# Autodesk Inventor assembly: 1050.000(1)
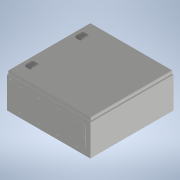
[picture p0: Inventor's stored thumbnail of the model, 180x180]
Saved by Autodesk Inventor 2021 (Build 250183000, 183)
## iProperties
Category: PARTsolutions
Company: RITTAL
Created: 2025-07-29
Part Number: 1050.000(1)
Catalog Web Link: www.cadenas.de
Description: AX Compact enclosure-sheet steel
Vendor: RITTAL
Document SubType Name: Assembly
Designer: psAdmin
Manufacturer: RITTAL
Mass: 2069.6 g
Surface Area: 25440.2 cm^2
Volume: 2069.6 cm^3
Density: 1 g/cm^3
Title: 1050.000(1)
Author: Cadenas PARTsolutions
Comments: sheet steel
PSOL_IDENT_0: {$CADENAS_DATA/23d-libs/rittal/schaltschranksys/kompakt_schaltschr/ae_2_0_asmtab.prj},203 {VTYP=3D},
PSOL_IDENT_1: {STYP=ASSTAB},{NB=1050.000(1)},{LINA=1050.000(1)},{NN=AX Compact enclosure},{DATE=28.04.2025 21:11:2
PSOL_IDENT_2: 3},{GEOMDATE=11.04.2025 11:21:44},{VERSION=},{LINEID=180},{WBVAR=DETAIL},{WBNUMERIC=DETAIL}  {NB=105
PSOL_IDENT_3: 0.000(1)},{LINA=1050.000(1)},{KT=DUMMY},{BEST=1050.000},{BEM=2},{DETAIL=1},{INFOWWW=Website},{BEZ1=A
PSOL_IDENT_4: X Kompakt-Schaltschrank},{BEZ2=Stahlblech},{BEZ3=eintürig},{INFO=Überarbeitete Version 11/2024},{B=5
PSOL_IDENT_5: 00},{H=500},{T=210},{F=450},{G=475},{B1=500},{H1=500},{T1=210},{F1=450},{G1=475},{S=2.5},{ST=MIN},{G
PSOL_IDENT_6: EW=15,42},{VERS=13},{CNSECLASS51=27-18-01-02},{CNSECLASS70=27-18-01-01},{CNSECLASS80=27-18-01-01},{C
PSOL_IDENT_7: NSETIM40=EC000261},{PPATH=assemblies_ae_2_0/ae_2_0_asmtpl.prj},{INFOPAGE=ax_s30},{INFOPATH=http://ww
PSOL_IDENT_8: w.rittal.com/com-en/part/1050000},{BESTE1=1050},{BESTE2=000},{DETAIL1= 2, 'niedrig', 'detail_2.png',
PSOL_IDENT_9: 1, 'hoch', 'detail_1.png', 11  , 'hochsperr', 'detail_11.png'},{CNSETIM80=EC000261},{CNSETIM90=EC00
PSOL_IDENT_10: 0261},{CNSECLASS60=27-18-01-01},{UNSPSC=31-26-15-02}
NB: 1050.000(1)
NN: AX Compact enclosure
NT: sheet steel
NBSYN: $BEST.($DETAIL.)
LINA: 1050.000(1)
CATALOG: Rittal
BEST: 1050.000
DETAIL: high
INFOWWW: webseite
BEZ1: AX Compact enclosure
BEZ2: sheet steel
BEZ3: single door
INFO: Revised version 11/2024
B: 500
H: 500
T: 210
F: 450
G: 475
GEW: 15,42
CNSECLASS70: 27-18-01-01
CNSECLASS80: 27-18-01-01
CNSETIM80: EC000261
CNSETIM90: EC000261
CNSECLASS60: 27-18-01-01
UNSPSC: 31-26-15-02
SUPPLIER: RITTAL
ARTICLENO: 1050.000(1)
BOMINFO: 1050.000(1)
CREATOR: CADENAS GmbH
## Documents named in this file (13)
- e:\temp\worker_COMMON_111\temp\tmp_7988_54_uwvFr\format_0\1050_000(1).iam
- e:\temp\worker_COMMON_111\temp\tmp_7988_54_uwvFr\format_0\1050_000(1)_P1.ipt
- e:\temp\worker_COMMON_111\temp\tmp_7988_54_uwvFr\format_0\1XXX_01_04(B,1)_P7.ipt
- e:\temp\worker_COMMON_111\temp\tmp_7988_54_uwvFr\format_0\1XXX_01_04(T,1)_P7.ipt
- e:\temp\worker_COMMON_111\temp\tmp_7988_54_uwvFr\format_0\155X_01_01(1)_P2.ipt
- e:\temp\worker_COMMON_111\temp\tmp_7988_54_uwvFr\format_0\6321_050_P9 1.ipt
- e:\temp\worker_COMMON_111\temp\tmp_7988_54_uwvFr\format_0\1XXX_01_05(1)_P8.ipt
- e:\temp\worker_COMMON_111\temp\tmp_7988_54_uwvFr\format_0\0000-00186369(1).ipt
- e:\temp\worker_COMMON_111\temp\tmp_7988_54_uwvFr\format_0\1XX4_04_00_4(1)_P5.ipt
- e:\temp\worker_COMMON_111\temp\tmp_7988_54_uwvFr\format_0\0000-00082819_P2.ipt
- e:\temp\worker_COMMON_111\temp\tmp_7988_54_uwvFr\format_0\155X_02_00_P6_(1).ipt
- e:\temp\worker_COMMON_111\temp\tmp_7988_54_uwvFr\format_0\0000-00168553(1).ipt
- e:\temp\worker_COMMON_111\temp\tmp_7988_54_uwvFr\format_0\0000-00189079(1).ipt
## Components (26 placed, 12 different names)
1. 1050_000(1)_P1:1 — SCRO_XY@1 <-> SC_XY@2, SCRO_Z@1 <-> SC_Z@2, SCRO_YZ@1 <-> SC_YZ@2, SCRU_XY@1 <-> SC_XY@3, SCRU_Z@1 <-> SC_Z@3, SCRU_YZ@1 <-> SC_YZ@3, SCLO_XY@1 <-> Hinge_Plug_XY@8, SCLO_Z@1 <-> Hinge_Plug_Z@8, SCLO_YZ@1 <-> Hinge_Plug_YZ@8, SCLU_XY@1 <-> Hinge_Plug_XY@9, SCLU_Z@1 <-> Hinge_Plug_Z@9, SCLU_YZ@1 <-> Hinge_Plug_YZ@9, FP1_XY@1 <-> FP_XY@10, FP1_Z@1 <-> FP_Z@10, FP1_YZ@1 <-> FP_YZ@10, MP_XY@1 <-> MP_XY@21, MP_Z@1 <-> MP_Z@21, MP_YZ@1 <-> MP_YZ@21, to_Plug_XY@1 <-> P1_XY@22, to_Plug_Z@1 <-> P1_Z@22, to_Plug_YZ@1 <-> P1_YZ@22, to_Cap_1_XY@1 <-> CAP_XY@23, to_Cap_1_Z@1 <-> CAP_Z@23, to_Cap_1_YZ@1 <-> CAP_YZ@23, to_Cap_2_XY@1 <-> CAP_XY@24, to_Cap_2_Z@1 <-> CAP_Z@24, to_Cap_2_YZ@1 <-> CAP_YZ@24, to_Cap_3_XY@1 <-> CAP_XY@25, to_Cap_3_Z@1 <-> CAP_Z@25, to_Cap_3_YZ@1 <-> CAP_YZ@25, to_Cap_4_XY@1 <-> CAP_XY@26, to_Cap_4_Z@1 <-> CAP_Z@26, to_Cap_4_YZ@1 <-> CAP_YZ@26
2. 1XXX_01_04(B,1)_P7:1 — SCRO_XY@1 <-> SC_XY@2, SCRO_Z@1 <-> SC_Z@2, SCRO_YZ@1 <-> SC_YZ@2
3. 1XXX_01_04(T,1)_P7:1 — SCRU_XY@1 <-> SC_XY@3, SCRU_Z@1 <-> SC_Z@3, SCRU_YZ@1 <-> SC_YZ@3, TUER2_XY@3 <-> ET_XY@4, TUER2_Z@3 <-> ET_Z@4
4. 155X_01_01(1)_P2:1 — TUER2_XY@3 <-> ET_XY@4, TUER2_Z@3 <-> ET_Z@4, to_Auflaufelement_XY@4 <-> P9_XY@5, to_Auflaufelement_Z@4 <-> P9_Z@5, to_Auflaufelement_YZ@4 <-> P9_YZ@5, VV1_XY@4 <-> VV_XY@6, VV1_Z@4 <-> VV_Z@6, VV1_YZ@4 <-> VV_YZ@6, VV2_XY@4 <-> VV_XY@7, VV2_Z@4 <-> VV_Z@7, VV2_YZ@4 <-> VV_YZ@7
5. 6321_050_P9 1:1 — to_Auflaufelement_XY@4 <-> P9_XY@5, to_Auflaufelement_Z@4 <-> P9_Z@5, to_Auflaufelement_YZ@4 <-> P9_YZ@5
6. 1XXX_01_05(1)_P8:1 — VV1_XY@4 <-> VV_XY@6, VV1_Z@4 <-> VV_Z@6, VV1_YZ@4 <-> VV_YZ@6
7. 1XXX_01_05(1)_P8:2 — VV2_XY@4 <-> VV_XY@7, VV2_Z@4 <-> VV_Z@7, VV2_YZ@4 <-> VV_YZ@7
8. 0000-00186369(1):1 — SCLO_XY@1 <-> Hinge_Plug_XY@8, SCLO_Z@1 <-> Hinge_Plug_Z@8, SCLO_YZ@1 <-> Hinge_Plug_YZ@8
9. 0000-00186369(1):2 — SCLU_XY@1 <-> Hinge_Plug_XY@9, SCLU_Z@1 <-> Hinge_Plug_Z@9, SCLU_YZ@1 <-> Hinge_Plug_YZ@9
10. 1XX4_04_00_4(1)_P5:1 — FP1_XY@1 <-> FP_XY@10, FP1_Z@1 <-> FP_Z@10, FP1_YZ@1 <-> FP_YZ@10, to_Bolt_1_XY@10 <-> Bolt_XY@11, to_Bolt_1_Z@10 <-> Bolt_Z@11, to_Bolt_1_YZ@10 <-> Bolt_YZ@11, to_Bolt_2_XY@10 <-> Bolt_XY@12, to_Bolt_2_Z@10 <-> Bolt_Z@12, to_Bolt_2_YZ@10 <-> Bolt_YZ@12, to_Bolt_1_1_XY@10 <-> Bolt_XY@13, to_Bolt_1_1_Z@10 <-> Bolt_Z@13, to_Bolt_1_1_YZ@10 <-> Bolt_YZ@13, to_Bolt_1_2_XY@10 <-> Bolt_XY@14, to_Bolt_1_2_Z@10 <-> Bolt_Z@14, to_Bolt_1_2_YZ@10 <-> Bolt_YZ@14, to_Bolt_1_3_XY@10 <-> Bolt_XY@15, to_Bolt_1_3_Z@10 <-> Bolt_Z@15, to_Bolt_1_3_YZ@10 <-> Bolt_YZ@15, to_Bolt_1_4_XY@10 <-> Bolt_XY@16, to_Bolt_1_4_Z@10 <-> Bolt_Z@16, to_Bolt_1_4_YZ@10 <-> Bolt_YZ@16, to_Bolt_1_5_XY@10 <-> Bolt_XY@17, to_Bolt_1_5_Z@10 <-> Bolt_Z@17, to_Bolt_1_5_YZ@10 <-> Bolt_YZ@17, to_Bolt_1_6_XY@10 <-> Bolt_XY@18, to_Bolt_1_6_Z@10 <-> Bolt_Z@18, to_Bolt_1_6_YZ@10 <-> Bolt_YZ@18, to_Bolt_1_7_XY@10 <-> Bolt_XY@19, to_Bolt_1_7_Z@10 <-> Bolt_Z@19, to_Bolt_1_7_YZ@10 <-> Bolt_YZ@19, to_Bolt_1_8_XY@10 <-> Bolt_XY@20, to_Bolt_1_8_Z@10 <-> Bolt_Z@20, to_Bolt_1_8_YZ@10 <-> Bolt_YZ@20
11. 0000-00082819_P2:1 — to_Bolt_1_XY@10 <-> Bolt_XY@11, to_Bolt_1_Z@10 <-> Bolt_Z@11, to_Bolt_1_YZ@10 <-> Bolt_YZ@11
12. 0000-00082819_P2:2 — to_Bolt_2_XY@10 <-> Bolt_XY@12, to_Bolt_2_Z@10 <-> Bolt_Z@12, to_Bolt_2_YZ@10 <-> Bolt_YZ@12
13. 0000-00082819_P2:3 — to_Bolt_1_1_XY@10 <-> Bolt_XY@13, to_Bolt_1_1_Z@10 <-> Bolt_Z@13, to_Bolt_1_1_YZ@10 <-> Bolt_YZ@13
14. 0000-00082819_P2:4 — to_Bolt_1_2_XY@10 <-> Bolt_XY@14, to_Bolt_1_2_Z@10 <-> Bolt_Z@14, to_Bolt_1_2_YZ@10 <-> Bolt_YZ@14
15. 0000-00082819_P2:5 — to_Bolt_1_3_XY@10 <-> Bolt_XY@15, to_Bolt_1_3_Z@10 <-> Bolt_Z@15, to_Bolt_1_3_YZ@10 <-> Bolt_YZ@15
16. 0000-00082819_P2:6 — to_Bolt_1_4_XY@10 <-> Bolt_XY@16, to_Bolt_1_4_Z@10 <-> Bolt_Z@16, to_Bolt_1_4_YZ@10 <-> Bolt_YZ@16
17. 0000-00082819_P2:7 — to_Bolt_1_5_XY@10 <-> Bolt_XY@17, to_Bolt_1_5_Z@10 <-> Bolt_Z@17, to_Bolt_1_5_YZ@10 <-> Bolt_YZ@17
18. 0000-00082819_P2:8 — to_Bolt_1_6_XY@10 <-> Bolt_XY@18, to_Bolt_1_6_Z@10 <-> Bolt_Z@18, to_Bolt_1_6_YZ@10 <-> Bolt_YZ@18
19. 0000-00082819_P2:9 — to_Bolt_1_7_XY@10 <-> Bolt_XY@19, to_Bolt_1_7_Z@10 <-> Bolt_Z@19, to_Bolt_1_7_YZ@10 <-> Bolt_YZ@19
20. 0000-00082819_P2:10 — to_Bolt_1_8_XY@10 <-> Bolt_XY@20, to_Bolt_1_8_Z@10 <-> Bolt_Z@20, to_Bolt_1_8_YZ@10 <-> Bolt_YZ@20
21. 155X_02_00_P6_(1):1 — MP_XY@1 <-> MP_XY@21, MP_Z@1 <-> MP_Z@21, MP_YZ@1 <-> MP_YZ@21
22. 0000-00168553(1):1 — to_Plug_XY@1 <-> P1_XY@22, to_Plug_Z@1 <-> P1_Z@22, to_Plug_YZ@1 <-> P1_YZ@22
23. 0000-00189079(1):1 — to_Cap_1_XY@1 <-> CAP_XY@23, to_Cap_1_Z@1 <-> CAP_Z@23, to_Cap_1_YZ@1 <-> CAP_YZ@23
24. 0000-00189079(1):2 — to_Cap_2_XY@1 <-> CAP_XY@24, to_Cap_2_Z@1 <-> CAP_Z@24, to_Cap_2_YZ@1 <-> CAP_YZ@24
25. 0000-00189079(1):3 — to_Cap_3_XY@1 <-> CAP_XY@25, to_Cap_3_Z@1 <-> CAP_Z@25, to_Cap_3_YZ@1 <-> CAP_YZ@25
26. 0000-00189079(1):4 — to_Cap_4_XY@1 <-> CAP_XY@26, to_Cap_4_Z@1 <-> CAP_Z@26, to_Cap_4_YZ@1 <-> CAP_YZ@26
## Relationships (74: Mate 49, Angle 24, Flush 1)
- SCRO_XY@1 <-> SC_XY@2 [Mate]: 1050_000(1)_P1:1 ↔ 1XXX_01_04(B,1)_P7:1
- SCRO_Z@1 <-> SC_Z@2 [Mate]: 1050_000(1)_P1:1 ↔ 1XXX_01_04(B,1)_P7:1
- SCRO_YZ@1 <-> SC_YZ@2 [Angle] (0 deg): 1050_000(1)_P1:1 ↔ 1XXX_01_04(B,1)_P7:1
- SCRU_XY@1 <-> SC_XY@3 [Mate]: 1050_000(1)_P1:1 ↔ 1XXX_01_04(T,1)_P7:1
- SCRU_Z@1 <-> SC_Z@3 [Mate]: 1050_000(1)_P1:1 ↔ 1XXX_01_04(T,1)_P7:1
- SCRU_YZ@1 <-> SC_YZ@3 [Angle] (0 deg): 1050_000(1)_P1:1 ↔ 1XXX_01_04(T,1)_P7:1
- TUER2_XY@3 <-> ET_XY@4 [Mate]: 1XXX_01_04(T,1)_P7:1 ↔ 155X_01_01(1)_P2:1
- TUER2_Z@3 <-> ET_Z@4 [Mate]: 1XXX_01_04(T,1)_P7:1 ↔ 155X_01_01(1)_P2:1
- to_Auflaufelement_XY@4 <-> P9_XY@5 [Mate]: 155X_01_01(1)_P2:1 ↔ 6321_050_P9 1:1
- to_Auflaufelement_Z@4 <-> P9_Z@5 [Mate]: 155X_01_01(1)_P2:1 ↔ 6321_050_P9 1:1
- to_Auflaufelement_YZ@4 <-> P9_YZ@5 [Angle] (180 deg): 155X_01_01(1)_P2:1 ↔ 6321_050_P9 1:1
- VV1_XY@4 <-> VV_XY@6 [Mate]: 155X_01_01(1)_P2:1 ↔ 1XXX_01_05(1)_P8:1
- VV1_Z@4 <-> VV_Z@6 [Mate]: 155X_01_01(1)_P2:1 ↔ 1XXX_01_05(1)_P8:1
- VV1_YZ@4 <-> VV_YZ@6 [Angle] (0 deg): 155X_01_01(1)_P2:1 ↔ 1XXX_01_05(1)_P8:1
- VV2_XY@4 <-> VV_XY@7 [Mate]: 155X_01_01(1)_P2:1 ↔ 1XXX_01_05(1)_P8:2
- VV2_Z@4 <-> VV_Z@7 [Mate]: 155X_01_01(1)_P2:1 ↔ 1XXX_01_05(1)_P8:2
- VV2_YZ@4 <-> VV_YZ@7 [Angle] (0 deg): 155X_01_01(1)_P2:1 ↔ 1XXX_01_05(1)_P8:2
- SCLO_XY@1 <-> Hinge_Plug_XY@8 [Mate] (1.25 mm): 1050_000(1)_P1:1 ↔ 0000-00186369(1):1
- SCLO_Z@1 <-> Hinge_Plug_Z@8 [Mate]: 1050_000(1)_P1:1 ↔ 0000-00186369(1):1
- SCLO_YZ@1 <-> Hinge_Plug_YZ@8 [Angle] (0 deg): 1050_000(1)_P1:1 ↔ 0000-00186369(1):1
- SCLU_XY@1 <-> Hinge_Plug_XY@9 [Mate] (1.25 mm): 1050_000(1)_P1:1 ↔ 0000-00186369(1):2
- SCLU_Z@1 <-> Hinge_Plug_Z@9 [Mate]: 1050_000(1)_P1:1 ↔ 0000-00186369(1):2
- SCLU_YZ@1 <-> Hinge_Plug_YZ@9 [Angle] (0 deg): 1050_000(1)_P1:1 ↔ 0000-00186369(1):2
- FP1_XY@1 <-> FP_XY@10 [Mate]: 1050_000(1)_P1:1 ↔ 1XX4_04_00_4(1)_P5:1
- FP1_Z@1 <-> FP_Z@10 [Mate]: 1050_000(1)_P1:1 ↔ 1XX4_04_00_4(1)_P5:1
- FP1_YZ@1 <-> FP_YZ@10 [Angle] (0 deg): 1050_000(1)_P1:1 ↔ 1XX4_04_00_4(1)_P5:1
- to_Bolt_1_XY@10 <-> Bolt_XY@11 [Mate]: 1XX4_04_00_4(1)_P5:1 ↔ 0000-00082819_P2:1
- to_Bolt_1_Z@10 <-> Bolt_Z@11 [Mate]: 1XX4_04_00_4(1)_P5:1 ↔ 0000-00082819_P2:1
- to_Bolt_1_YZ@10 <-> Bolt_YZ@11 [Angle] (0 deg): 1XX4_04_00_4(1)_P5:1 ↔ 0000-00082819_P2:1
- to_Bolt_2_XY@10 <-> Bolt_XY@12 [Mate]: 1XX4_04_00_4(1)_P5:1 ↔ 0000-00082819_P2:2
- to_Bolt_2_Z@10 <-> Bolt_Z@12 [Mate]: 1XX4_04_00_4(1)_P5:1 ↔ 0000-00082819_P2:2
- to_Bolt_2_YZ@10 <-> Bolt_YZ@12 [Angle] (0 deg): 1XX4_04_00_4(1)_P5:1 ↔ 0000-00082819_P2:2
- to_Bolt_1_1_XY@10 <-> Bolt_XY@13 [Mate]: 1XX4_04_00_4(1)_P5:1 ↔ 0000-00082819_P2:3
- to_Bolt_1_1_Z@10 <-> Bolt_Z@13 [Mate]: 1XX4_04_00_4(1)_P5:1 ↔ 0000-00082819_P2:3
- to_Bolt_1_1_YZ@10 <-> Bolt_YZ@13 [Angle] (0 deg): 1XX4_04_00_4(1)_P5:1 ↔ 0000-00082819_P2:3
- to_Bolt_1_2_XY@10 <-> Bolt_XY@14 [Mate]: 1XX4_04_00_4(1)_P5:1 ↔ 0000-00082819_P2:4
- to_Bolt_1_2_Z@10 <-> Bolt_Z@14 [Mate]: 1XX4_04_00_4(1)_P5:1 ↔ 0000-00082819_P2:4
- to_Bolt_1_2_YZ@10 <-> Bolt_YZ@14 [Angle] (0 deg): 1XX4_04_00_4(1)_P5:1 ↔ 0000-00082819_P2:4
- to_Bolt_1_3_XY@10 <-> Bolt_XY@15 [Mate]: 1XX4_04_00_4(1)_P5:1 ↔ 0000-00082819_P2:5
- to_Bolt_1_3_Z@10 <-> Bolt_Z@15 [Mate]: 1XX4_04_00_4(1)_P5:1 ↔ 0000-00082819_P2:5
- to_Bolt_1_3_YZ@10 <-> Bolt_YZ@15 [Angle] (0 deg): 1XX4_04_00_4(1)_P5:1 ↔ 0000-00082819_P2:5
- to_Bolt_1_4_XY@10 <-> Bolt_XY@16 [Mate]: 1XX4_04_00_4(1)_P5:1 ↔ 0000-00082819_P2:6
- to_Bolt_1_4_Z@10 <-> Bolt_Z@16 [Mate]: 1XX4_04_00_4(1)_P5:1 ↔ 0000-00082819_P2:6
- to_Bolt_1_4_YZ@10 <-> Bolt_YZ@16 [Angle] (0 deg): 1XX4_04_00_4(1)_P5:1 ↔ 0000-00082819_P2:6
- to_Bolt_1_5_XY@10 <-> Bolt_XY@17 [Mate]: 1XX4_04_00_4(1)_P5:1 ↔ 0000-00082819_P2:7
- to_Bolt_1_5_Z@10 <-> Bolt_Z@17 [Mate]: 1XX4_04_00_4(1)_P5:1 ↔ 0000-00082819_P2:7
- to_Bolt_1_5_YZ@10 <-> Bolt_YZ@17 [Angle] (0 deg): 1XX4_04_00_4(1)_P5:1 ↔ 0000-00082819_P2:7
- to_Bolt_1_6_XY@10 <-> Bolt_XY@18 [Mate]: 1XX4_04_00_4(1)_P5:1 ↔ 0000-00082819_P2:8
- to_Bolt_1_6_Z@10 <-> Bolt_Z@18 [Mate]: 1XX4_04_00_4(1)_P5:1 ↔ 0000-00082819_P2:8
- to_Bolt_1_6_YZ@10 <-> Bolt_YZ@18 [Angle] (0 deg): 1XX4_04_00_4(1)_P5:1 ↔ 0000-00082819_P2:8
- to_Bolt_1_7_XY@10 <-> Bolt_XY@19 [Mate]: 1XX4_04_00_4(1)_P5:1 ↔ 0000-00082819_P2:9
- to_Bolt_1_7_Z@10 <-> Bolt_Z@19 [Mate]: 1XX4_04_00_4(1)_P5:1 ↔ 0000-00082819_P2:9
- to_Bolt_1_7_YZ@10 <-> Bolt_YZ@19 [Angle] (0 deg): 1XX4_04_00_4(1)_P5:1 ↔ 0000-00082819_P2:9
- to_Bolt_1_8_XY@10 <-> Bolt_XY@20 [Mate]: 1XX4_04_00_4(1)_P5:1 ↔ 0000-00082819_P2:10
- to_Bolt_1_8_Z@10 <-> Bolt_Z@20 [Mate]: 1XX4_04_00_4(1)_P5:1 ↔ 0000-00082819_P2:10
- to_Bolt_1_8_YZ@10 <-> Bolt_YZ@20 [Angle] (0 deg): 1XX4_04_00_4(1)_P5:1 ↔ 0000-00082819_P2:10
- MP_XY@1 <-> MP_XY@21 [Mate] (0.25 mm): 1050_000(1)_P1:1 ↔ 155X_02_00_P6_(1):1
- MP_Z@1 <-> MP_Z@21 [Mate]: 1050_000(1)_P1:1 ↔ 155X_02_00_P6_(1):1
- MP_YZ@1 <-> MP_YZ@21 [Angle] (0 deg): 1050_000(1)_P1:1 ↔ 155X_02_00_P6_(1):1
- to_Plug_XY@1 <-> P1_XY@22 [Flush]: 1050_000(1)_P1:1 ↔ 0000-00168553(1):1
- to_Plug_Z@1 <-> P1_Z@22 [Mate]: 1050_000(1)_P1:1 ↔ 0000-00168553(1):1
- to_Plug_YZ@1 <-> P1_YZ@22 [Angle] (0 deg): 1050_000(1)_P1:1 ↔ 0000-00168553(1):1
- to_Cap_1_XY@1 <-> CAP_XY@23 [Mate] (-1.55 mm): 1050_000(1)_P1:1 ↔ 0000-00189079(1):1
- to_Cap_1_Z@1 <-> CAP_Z@23 [Mate]: 1050_000(1)_P1:1 ↔ 0000-00189079(1):1
- to_Cap_1_YZ@1 <-> CAP_YZ@23 [Angle] (0 deg): 1050_000(1)_P1:1 ↔ 0000-00189079(1):1
- to_Cap_2_XY@1 <-> CAP_XY@24 [Mate] (-1.55 mm): 1050_000(1)_P1:1 ↔ 0000-00189079(1):2
- to_Cap_2_Z@1 <-> CAP_Z@24 [Mate]: 1050_000(1)_P1:1 ↔ 0000-00189079(1):2
- to_Cap_2_YZ@1 <-> CAP_YZ@24 [Angle] (0 deg): 1050_000(1)_P1:1 ↔ 0000-00189079(1):2
- to_Cap_3_XY@1 <-> CAP_XY@25 [Mate] (-1.55 mm): 1050_000(1)_P1:1 ↔ 0000-00189079(1):3
- to_Cap_3_Z@1 <-> CAP_Z@25 [Mate]: 1050_000(1)_P1:1 ↔ 0000-00189079(1):3
- to_Cap_3_YZ@1 <-> CAP_YZ@25 [Angle] (0 deg): 1050_000(1)_P1:1 ↔ 0000-00189079(1):3
- to_Cap_4_XY@1 <-> CAP_XY@26 [Mate] (-1.55 mm): 1050_000(1)_P1:1 ↔ 0000-00189079(1):4
- to_Cap_4_Z@1 <-> CAP_Z@26 [Mate]: 1050_000(1)_P1:1 ↔ 0000-00189079(1):4
- to_Cap_4_YZ@1 <-> CAP_YZ@26 [Angle] (0 deg): 1050_000(1)_P1:1 ↔ 0000-00189079(1):4
